# Autodesk Inventor assembly: Cabinet
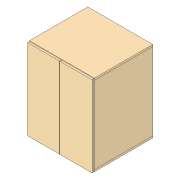
[picture p0: Inventor's stored thumbnail of the model, 180x180]
Saved by Autodesk Inventor 2022.1 (Build 261234020, 234B)
## iProperties
Created: 2022-05-10
Part Number: Cabinet
Document SubType Name: Assembly
Designer: sauliusd
Author: sauliusd
## iProperties of the stored document MemberDocs/xNfjotp5kDk1ezpyiVlelxpzoMh
RuleStatus: InUse
Created: 2022-05-10
Part Number: Cabinet
Document SubType Name: Assembly
Designer: sauliusd
Author: sauliusd
## iProperties of the stored document MemberDocs/x1gh1xroiCk5efnxdRoc1wo1lNb
RuleStatus: InUse
Created: 2022-05-10
Part Number: Cabinet
Document SubType Name: Assembly
Designer: sauliusd
Author: sauliusd
## Documents named in this file (52)
- C:\W4INV 2024 Design\PROJECTS\Samples\API Demo\Standing Cabinet\Cabinet.iam
- C:\W4INV 2022 Design\PROJECTS\Samples\API Samples\Stand Cabinet\Left Panel.ipt
- C:\W4INV 2022 Design\PROJECTS\Samples\API Samples\Stand Cabinet\Top Panel.ipt
- C:\W4INV 2022 Design\PROJECTS\Samples\API Samples\Stand Cabinet\Right Panel.ipt
- C:\W4INV 2022 Design\PROJECTS\Samples\API Samples\Stand Cabinet\Bottom Panel.ipt
- C:\W4INV 2022 Design\PROJECTS\Samples\API Samples\Stand Cabinet\Back Panel.ipt
- C:\W4INV 2022 Design\PROJECTS\Samples\API Samples\Stand Cabinet\Left Door.ipt
- C:\W4INV 2022 Design\PROJECTS\Samples\API Samples\Stand Cabinet\Right Door.ipt
- C:\W4INV 2022 Design\PROJECTS\Samples\API Samples\Stand Cabinet\Shelf.ipt
- C:\W4INV 2022 Design\PROJECTS\Samples\API Samples\Stand Cabinet\Door.ipt
- C:\W4INV 2022 Design\PROJECTS\Samples\API Samples\Stand Cabinet\Cabinet.ipt
- C:\W4INV 2024 Design\PROJECTS\Samples\API Demo\Standing Cabinet\Left Panel.ipt
- C:\W4INV 2024 Design\PROJECTS\Samples\API Demo\Standing Cabinet\Top Panel.ipt
- C:\W4INV 2024 Design\PROJECTS\Samples\API Demo\Standing Cabinet\Right Panel.ipt
- C:\W4INV 2024 Design\PROJECTS\Samples\API Demo\Standing Cabinet\Bottom Panel.ipt
- C:\W4INV 2024 Design\PROJECTS\Samples\API Demo\Standing Cabinet\Back Panel.ipt
- C:\W4INV 2024 Design\PROJECTS\Samples\API Demo\Standing Cabinet\Left Door.ipt
- C:\W4INV 2024 Design\PROJECTS\Samples\API Demo\Standing Cabinet\Right Door.ipt
- C:\W4INV 2024 Design\PROJECTS\Samples\API Demo\Standing Cabinet\Shelf.ipt
- C:\W4INV 2024 Design\PROJECTS\Samples\API Demo\Standing Cabinet\Door.ipt
- C:\W4INV 2024 Design\PROJECTS\Samples\API Demo\Standing Cabinet\Cabinet.ipt
- C:\W4INV 2024 Design\PROJECTS\Samples\API Demo\Standing Cabinet\Left Plynth.ipt
- C:\W4INV 2024 Design\PROJECTS\Samples\API Demo\Standing Cabinet\Front Plynth.ipt
- C:\W4INV 2024 Design\PROJECTS\Samples\API Demo\Standing Cabinet\Right Plynth.ipt
- C:\W4INV 2024 Design\PROJECTS\Samples\API Demo\Standing Cabinet\Back Plynth.ipt
- C:\W4INV 2024 Design\_LIBRARY\Hinges\CONCEALED HINGE\Full Overlay Hinge Wood Screw Cup Wood Screw T18.iam
- C:\W4INV 2022 Design\LIBRARY\Hinges\CONCEALED HINGE.iam
- C:\W4INV 2024 Design\PROJECTS\MODEL STATE LIBRARY COMPONENTS\Minifix D15\Minifix D15.iam
- C:\W4INV 2024 Design\_LIBRARY\Holders\Shelf holder D5\Shelf support D5 L16 with hole covers.ipt
- C:\W4INV 2022 Design\LIBRARY\Holders\Shelf holder D5.ipt
- C:\W4INV 2024 Design\PROJECTS\Samples\API Demo\Standing Cabinet\Handle.ipt
- C:\W4INV 2024 Design\_LIBRARY\Fixed joints\Dowel\DOWEL V2\Dowel 8x30 PB T=18.ipt
- C:\W4INV 2022 Design\LIBRARY\Fixed joints\Dowel\DOWEL V2.ipt
- C:\W4INV 2022 Design\PROJECTS\Samples\API Samples\Standing Cabinet\Left Panel.ipt
- C:\W4INV 2022 Design\PROJECTS\Samples\API Samples\Standing Cabinet\Top Panel.ipt
- C:\W4INV 2022 Design\PROJECTS\Samples\API Samples\Standing Cabinet\Right Panel.ipt
- C:\W4INV 2022 Design\PROJECTS\Samples\API Samples\Standing Cabinet\Bottom Panel.ipt
- C:\W4INV 2022 Design\PROJECTS\Samples\API Samples\Standing Cabinet\Back Panel.ipt
- C:\W4INV 2022 Design\PROJECTS\Samples\API Samples\Standing Cabinet\Left Door.ipt
- C:\W4INV 2022 Design\PROJECTS\Samples\API Samples\Standing Cabinet\Right Door.ipt
- C:\W4INV 2022 Design\PROJECTS\Samples\API Samples\Standing Cabinet\Shelf.ipt
- C:\W4INV 2022 Design\PROJECTS\Samples\API Samples\Standing Cabinet\Door.ipt
- C:\W4INV 2022 Design\PROJECTS\Samples\API Samples\Standing Cabinet\Cabinet.ipt
- C:\W4INV 2022 Design\PROJECTS\Samples\API Samples\Standing Cabinet\Left Plynth.ipt
- C:\W4INV 2022 Design\PROJECTS\Samples\API Samples\Standing Cabinet\Front Plynth.ipt
- C:\W4INV 2022 Design\PROJECTS\Samples\API Samples\Standing Cabinet\Right Plynth.ipt
- C:\W4INV 2022 Design\PROJECTS\Samples\API Samples\Standing Cabinet\Back Plynth.ipt
- C:\W4INV 2022 Design\_LIBRARY\Hinges\CONCEALED HINGE\Full Overlay Hinge Wood Screw Cup Wood Screw T18.iam
- C:\W4INV 2022 Design\PROJECTS\MODEL STATE LIBRARY COMPONENTS\Minifix D15\Minifix D15.iam
- C:\W4INV 2022 Design\_LIBRARY\Holders\Shelf holder D5\Shelf support D5 L16 with hole covers.ipt
- C:\W4INV 2022 Design\PROJECTS\Samples\API Samples\Standing Cabinet\Handle.ipt
- C:\W4INV 2022 Design\_LIBRARY\Fixed joints\Dowel\DOWEL V2\Dowel 8x30 PB T=18.ipt
## Components (10 placed, 10 different names)
1. @Skeleton — Flush:1, Flush:2, Flush:3
2. Left Panel:1
3. Top Panel:1
4. Right Panel:1
5. Bottom Panel:1
6. Back Panel:1
7. Left Door:1
8. Right Door:1
9. Shelf:1
10. Door:1
## Relationships (3: Flush 3)
- Flush:1: @Skeleton
- Flush:2: @Skeleton
- Flush:3: @Skeleton
